# Autodesk Inventor assembly: dual_extruder_carryage
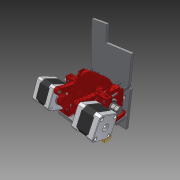
[picture p0: Inventor's stored thumbnail of the model, 180x180]
Saved by Autodesk Inventor 2014 (Build 180170000, 170)
## iProperties
Created: 2014-02-23
Part Number: dual_extruder_carryage
Document SubType Name: Assembly
Designer: buben
Author: buben
## Documents named in this file (6)
- C:\Users\buben\Documents\GitHub\bacon\inventor files\__concepts\dual_extruder_carryage.iam
- C:\Users\buben\Documents\GitHub\bacon\inventor files\__concepts\x_carriage_front.ipt
- C:\Users\buben\Documents\GitHub\bacon\inventor files\__concepts\x_carryage_extruder_mount.ipt
- C:\Users\buben\Documents\GitHub\bacon\inventor files\assemblies\dual_extruder.iam
- C:\Users\buben\Documents\GitHub\bacon\inventor files\3rd party components\linear_bearing_8\Imported Components\LU8MM\LU8MM.iam
- C:\Users\buben\Documents\GitHub\bacon\inventor files\__concepts\x_carryage_brace.ipt
## Components (7 placed, 5 different names)
1. x_carriage_front:1 — Mate:1, Flush:1, Mate:4, Mate:5, Mate:6, Mate:7, Mate:8, Mate:9, Mate:10, Mate:11, Mate:12, Mate:13, Mate:14, Mate:15, Mate:16, Mate:18
2. x_carryage_extruder_mount:1 — Mate:1, Flush:1, Mate:2, Angle:1, Mate:3, Mate:16, Mate:17, Mate:19
3. dual_extruder:1 [sub-assembly] — Mate:2, Angle:1, Mate:3
4. LU8MM:1 [sub-assembly] — Mate:7, Mate:8, Mate:14
5. LU8MM:2 [sub-assembly] — Mate:9, Mate:10, Mate:15
6. LU8MM:3 [sub-assembly] — Mate:11, Mate:12, Mate:13
7. x_carryage_brace:1 — Mate:17, Mate:18, Mate:19
## Relationships (21: Mate 19, Flush 1, Angle 1)
- Mate:1: x_carriage_front:1 ↔ x_carryage_extruder_mount:1
- Flush:1: x_carriage_front:1 ↔ x_carryage_extruder_mount:1
- Mate:2: x_carryage_extruder_mount:1 ↔ dual_extruder:1
- Angle:1 (0 deg): x_carryage_extruder_mount:1 ↔ dual_extruder:1
- Mate:3: x_carryage_extruder_mount:1 ↔ dual_extruder:1
- Mate:4: x_carriage_front:1
- Mate:5: x_carriage_front:1
- Mate:6: x_carriage_front:1
- Mate:7 (7.5 mm): x_carriage_front:1 ↔ LU8MM:1
- Mate:8 (7.5 mm): x_carriage_front:1 ↔ LU8MM:1
- Mate:9 (7.5 mm): x_carriage_front:1 ↔ LU8MM:2
- Mate:10 (7.5 mm): x_carriage_front:1 ↔ LU8MM:2
- Mate:11 (7.5 mm): x_carriage_front:1 ↔ LU8MM:3
- Mate:12 (7.5 mm): x_carriage_front:1 ↔ LU8MM:3
- Mate:13 (0.5 mm): x_carriage_front:1 ↔ LU8MM:3
- Mate:14 (0.5 mm): x_carriage_front:1 ↔ LU8MM:1
- Mate:15 (0.5 mm): x_carriage_front:1 ↔ LU8MM:2
- Mate:16: x_carriage_front:1 ↔ x_carryage_extruder_mount:1
- Mate:17: x_carryage_extruder_mount:1 ↔ x_carryage_brace:1
- Mate:18: x_carriage_front:1 ↔ x_carryage_brace:1
- Mate:19: x_carryage_extruder_mount:1 ↔ x_carryage_brace:1
